# Autodesk Inventor assembly: MainStanokLathe
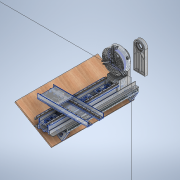
[picture p0: Inventor's stored thumbnail of the model, 180x180]
Saved by Autodesk Inventor 2022 (Build 260153000, 153)
## iProperties
Created: 2023-08-15
Part Number: MainStanokLathe
Document SubType Name: Assembly
Designer: Kippi
Mass: 47808.8 g
Surface Area: 40542.6 cm^2
Volume: 14656.1 cm^3
Density: 3.26205 g/cm^3
Author: Kippi
## Documents named in this file (11)
- C:\Users\Kippi\Documents\CNC_Lathe\MainStanokLathe.iam
- C:\Users\Kippi\Documents\CNC_Lathe\Stanina.iam
- C:\Users\Kippi\Documents\CNC_Lathe\YaxisAss.iam
- C:\Users\Kippi\Documents\CNC_Lathe\Rails\HGR20R LINEAR GUIDE RAIL, CONFIGURABLE, 1000 mm.ipt
- C:\Users\Kippi\Documents\CNC_Lathe\Rails\HGH20CAZ0C, BLOCK, MIDSECTION.ipt
- C:\Users\Kippi\Documents\CNC_Lathe\Podkladka.ipt
- C:\Users\Kippi\Documents\CNC_Lathe\FlanecForwardBabka.ipt
- C:\Users\Kippi\Documents\CNC_Lathe\Babka.iam
- C:\Users\Kippi\Documents\CNC_Lathe\KaretkaYaxis.ipt
- C:\Users\Kippi\Documents\CNC_Lathe\ProkladkaA.ipt
- C:\Users\Kippi\Documents\CNC_Lathe\KorpusOsnova.ipt
## Components (15 placed, 10 different names)
1. Stanina:1 [sub-assembly] — Mate:1, Mate:2, Flush:1, Flush:2, Flush:3, Flush:4, Flush:7, Mate:15, Mate:16, Mate:21, Mate:24, Mate:25, Mate:26
2. YaxisAss:1 [sub-assembly] — Mate:11, Flush:5, Mate:13, Mate:14, Mate:19
3. HGR20R LINEAR GUIDE RAIL, CONFIGURABLE, 1000 mm:1 — Mate:2, Flush:1, Flush:4, Mate:5, Mate:6, Mate:7, Mate:8
4. HGR20R LINEAR GUIDE RAIL, CONFIGURABLE, 1000 mm:2 — Mate:1, Flush:2, Flush:3, Mate:3, Mate:4, Mate:9, Mate:10
5. HGH20CAZ0C, BLOCK, MIDSECTION:1 — Mate:4, Mate:9
6. HGH20CAZ0C, BLOCK, MIDSECTION:2 — Mate:5, Mate:8
7. HGH20CAZ0C, BLOCK, MIDSECTION:3 — Mate:3, Mate:10
8. HGH20CAZ0C, BLOCK, MIDSECTION:4 — Mate:6, Mate:7, Mate:12, Flush:6
9. Podkladka:1 — Mate:11, Flush:5, Mate:12, Flush:6
10. HGH20CAZ0C, BLOCK, MIDSECTION:5 — Mate:13, Mate:14, Mate:20
11. FlanecForwardBabka:1 — Flush:7, Mate:15, Mate:16, Mate:22, Flush:8
12. KaretkaYaxis:2 — Mate:19, Mate:20
13. Babka:2 [sub-assembly] — Mate:23, Mate:24
14. ProkladkaA:2 — Mate:21, Mate:22, Flush:8, Mate:23
15. KorpusOsnova:2 — Mate:25, Mate:26
## Relationships (32: Mate 24, Flush 8)
- Mate:1: Stanina:1 ↔ HGR20R LINEAR GUIDE RAIL, CONFIGURABLE, 1000 mm:2
- Mate:2: Stanina:1 ↔ HGR20R LINEAR GUIDE RAIL, CONFIGURABLE, 1000 mm:1
- Flush:1: Stanina:1 ↔ HGR20R LINEAR GUIDE RAIL, CONFIGURABLE, 1000 mm:1
- Flush:2: Stanina:1 ↔ HGR20R LINEAR GUIDE RAIL, CONFIGURABLE, 1000 mm:2
- Flush:3: Stanina:1 ↔ HGR20R LINEAR GUIDE RAIL, CONFIGURABLE, 1000 mm:2
- Flush:4: Stanina:1 ↔ HGR20R LINEAR GUIDE RAIL, CONFIGURABLE, 1000 mm:1
- Mate:3: HGR20R LINEAR GUIDE RAIL, CONFIGURABLE, 1000 mm:2 ↔ HGH20CAZ0C, BLOCK, MIDSECTION:3
- Mate:4: HGR20R LINEAR GUIDE RAIL, CONFIGURABLE, 1000 mm:2 ↔ HGH20CAZ0C, BLOCK, MIDSECTION:1
- Mate:5: HGR20R LINEAR GUIDE RAIL, CONFIGURABLE, 1000 mm:1 ↔ HGH20CAZ0C, BLOCK, MIDSECTION:2
- Mate:6: HGR20R LINEAR GUIDE RAIL, CONFIGURABLE, 1000 mm:1 ↔ HGH20CAZ0C, BLOCK, MIDSECTION:4
- Mate:7: HGR20R LINEAR GUIDE RAIL, CONFIGURABLE, 1000 mm:1 ↔ HGH20CAZ0C, BLOCK, MIDSECTION:4
- Mate:8: HGR20R LINEAR GUIDE RAIL, CONFIGURABLE, 1000 mm:1 ↔ HGH20CAZ0C, BLOCK, MIDSECTION:2
- Mate:9: HGR20R LINEAR GUIDE RAIL, CONFIGURABLE, 1000 mm:2 ↔ HGH20CAZ0C, BLOCK, MIDSECTION:1
- Mate:10: HGR20R LINEAR GUIDE RAIL, CONFIGURABLE, 1000 mm:2 ↔ HGH20CAZ0C, BLOCK, MIDSECTION:3
- Mate:11: YaxisAss:1 ↔ Podkladka:1
- Flush:5: YaxisAss:1 ↔ Podkladka:1
- Mate:12: HGH20CAZ0C, BLOCK, MIDSECTION:4 ↔ Podkladka:1
- Flush:6: HGH20CAZ0C, BLOCK, MIDSECTION:4 ↔ Podkladka:1
- Mate:13: YaxisAss:1 ↔ HGH20CAZ0C, BLOCK, MIDSECTION:5
- Mate:14: YaxisAss:1 ↔ HGH20CAZ0C, BLOCK, MIDSECTION:5
- Flush:7: Stanina:1 ↔ FlanecForwardBabka:1
- Mate:15: Stanina:1 ↔ FlanecForwardBabka:1
- Mate:16: Stanina:1 ↔ FlanecForwardBabka:1
- Mate:19: YaxisAss:1 ↔ KaretkaYaxis:2
- Mate:20: HGH20CAZ0C, BLOCK, MIDSECTION:5 ↔ KaretkaYaxis:2
- Mate:21: Stanina:1 ↔ ProkladkaA:2
- Mate:22: FlanecForwardBabka:1 ↔ ProkladkaA:2
- Flush:8: FlanecForwardBabka:1 ↔ ProkladkaA:2
- Mate:23: Babka:2 ↔ ProkladkaA:2
- Mate:24: Stanina:1 ↔ Babka:2
- Mate:25: Stanina:1 ↔ KorpusOsnova:2
- Mate:26: Stanina:1 ↔ KorpusOsnova:2
